# Autodesk Inventor assembly: 8_Omni-Directional_Wheel_217-2613
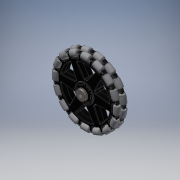
[picture p0: Inventor's stored thumbnail of the model, 180x180]
Saved by Autodesk Inventor 2018 (Build 220112000, 112)
## iProperties
Company: Microsoft
Created: 2012-12-03
Part Number: 8_Omni-Directional_Wheel_217-2613
Description: STEP AP203
Document SubType Name: Assembly
Designer: maste
Sending System: SolidWorks 2012
Preprocessor: SwSTEP 2.0
Title: 217-2613.20121203.STEP
Author: svradm
Revision Number: ANY
## Documents named in this file (12)
- C:\Users\maste\OneDrive\Documents\GitHub\2020CAD (offseason)\The Chad Kiwi\Part Files\8_Omni-Directional_Wheel_217-2613.iam
- C:\Users\maste\OneDrive\Documents\GitHub\2020CAD (offseason)\The Chad Kiwi\Part Files\217-2613-001 Rev1.ipt
- C:\Users\maste\OneDrive\Documents\GitHub\2020CAD (offseason)\The Chad Kiwi\Part Files\217-2613-003 Rev1.ipt
- C:\Users\maste\OneDrive\Documents\GitHub\2020CAD (offseason)\The Chad Kiwi\Part Files\217-2613-002 Rev1.ipt
- C:\Users\maste\OneDrive\Documents\GitHub\2020CAD (offseason)\The Chad Kiwi\Part Files\217-2613-004 Rev1.ipt
- C:\Users\maste\OneDrive\Documents\GitHub\2020CAD (offseason)\The Chad Kiwi\Part Files\BEAM-0750.ipt
- C:\Users\maste\OneDrive\Documents\GitHub\2020CAD (offseason)\The Chad Kiwi\Part Files\90116A020_90116A020.ipt
- C:\Users\maste\OneDrive\Documents\GitHub\2020CAD (offseason)\The Chad Kiwi\Part Files\217-2584-005 Rev1 A.ipt
- C:\Users\maste\OneDrive\Documents\GitHub\2020CAD (offseason)\The Chad Kiwi\Part Files\1_2_Hex_Bore_Aluminum_VersaHub_217-2592.ipt
- C:\Users\maste\OneDrive\Documents\GitHub\2020CAD (offseason)\The Chad Kiwi\Part Files\0.125 spacer.ipt
- C:\Users\maste\OneDrive\Documents\GitHub\2020CAD (offseason)\The Chad Kiwi\Part Files\0_500_Hex_ID_x_1_125_OD_x_0_313_WD_Flanged_Bearing_v2_217-3875.ipt
- C:\Users\maste\OneDrive\Documents\GitHub\2020CAD (offseason)\The Chad Kiwi\Part Files\am-1526 500Hex HD Collar Clamp (1).iam
## Components (114 placed, 113 different names)
1. 217-2613-001 Rev1_1
2. 217-2613-003 Rev1_2
3. 217-2613-002 Rev1_3 — Mate:4, Mate:5, Mate:6
4. 217-2613-001 Rev1_4
5. 217-2613-001 Rev1_5
6. 217-2613-001 Rev1_6
7. 217-2613-001 Rev1_7
8. 217-2613-001 Rev1_8
9. 217-2613-001 Rev1_9
10. 217-2613-001 Rev1_10
11. 217-2613-001 Rev1_11
12. 217-2613-001 Rev1_12
13. 217-2613-001 Rev1_13
14. 217-2613-001 Rev1_14
15. 217-2613-001 Rev1_15
16. 217-2613-001 Rev1_16
17. 217-2613-001 Rev1_17
18. 217-2613-001 Rev1_18
19. 217-2613-004 Rev1_19
20. 217-2613-004 Rev1_20
21. 217-2613-004 Rev1_21
22. 217-2613-004 Rev1_22
23. 217-2613-004 Rev1_23
24. 217-2613-004 Rev1_24
25. 217-2613-004 Rev1_25
26. 217-2613-004 Rev1_26
27. 217-2613-004 Rev1_27
28. 217-2613-004 Rev1_28
29. 217-2613-004 Rev1_29
30. 217-2613-004 Rev1_30
31. 217-2613-004 Rev1_31
32. 217-2613-004 Rev1_32
33. 217-2613-004 Rev1_33
34. 217-2613-004 Rev1_34
35. 217-2613-002 Rev1_35 — Mate:1, Mate:2, Mate:3
36. 217-2613-001 Rev1_36
37. 217-2613-004 Rev1_37
38. 217-2613-001 Rev1_38
39. 217-2613-001 Rev1_39
40. 217-2613-001 Rev1_40
41. 217-2613-001 Rev1_41
42. 217-2613-001 Rev1_42
43. 217-2613-001 Rev1_43
44. 217-2613-001 Rev1_44
45. 217-2613-001 Rev1_45
46. 217-2613-001 Rev1_46
47. 217-2613-001 Rev1_47
48. 217-2613-001 Rev1_48
49. 217-2613-001 Rev1_49
50. 217-2613-001 Rev1_50
51. 217-2613-001 Rev1_51
52. 217-2613-001 Rev1_52
53. 217-2613-004 Rev1_53
54. 217-2613-004 Rev1_54
55. 217-2613-004 Rev1_55
56. 217-2613-004 Rev1_56
57. 217-2613-004 Rev1_57
58. 217-2613-004 Rev1_58
59. 217-2613-004 Rev1_59
60. 217-2613-004 Rev1_60
61. 217-2613-004 Rev1_61
62. 217-2613-004 Rev1_62
63. 217-2613-004 Rev1_63
64. 217-2613-004 Rev1_64
65. 217-2613-004 Rev1_65
66. 217-2613-004 Rev1_66
67. 217-2613-004 Rev1_67
68. BEAM-0750_68
69. BEAM-0750_69
70. BEAM-0750_70
71. BEAM-0750_71
72. BEAM-0750_72
73. BEAM-0750_73
74. 90116A020_90116A020_74
75. 90116A020_90116A020_75
76. 90116A020_90116A020_76
77. 90116A020_90116A020_77
78. 90116A020_90116A020_78
79. 90116A020_90116A020_79
80. 90116A020_90116A020_80
81. 90116A020_90116A020_81
82. 90116A020_90116A020_82
83. 90116A020_90116A020_83
84. 90116A020_90116A020_84
85. 90116A020_90116A020_85
86. 90116A020_90116A020_86
87. 90116A020_90116A020_87
88. 90116A020_90116A020_88
89. 90116A020_90116A020_89
90. 90116A020_90116A020_90
91. 90116A020_90116A020_91
92. 90116A020_90116A020_92
93. 90116A020_90116A020_93
94. 90116A020_90116A020_94
95. 90116A020_90116A020_95
96. 90116A020_90116A020_96
97. 90116A020_90116A020_97
98. 90116A020_90116A020_98
99. 90116A020_90116A020_99
100. 90116A020_90116A020_100
101. 90116A020_90116A020_101
102. 90116A020_90116A020_102
103. 90116A020_90116A020_103
104. 90116A020_90116A020_104
105. 90116A020_90116A020_105
106. 217-2584-005 Rev1 A_106
107. 217-2584-005 Rev1 A_107
108. 217-2584-005 Rev1 A_108
109. 217-2584-005 Rev1 A_109
110. 1_2_Hex_Bore_Aluminum_VersaHub_217-2592:1 — Mate:1, Mate:2, Mate:3, Flush:1, Flush:2, Mate:7
111. 1_2_Hex_Bore_Aluminum_VersaHub_217-2592:2 — Mate:4, Mate:5, Mate:6, Flush:3, Flush:4, Mate:8
112. 0.125 spacer:1 — Flush:3, Flush:4, Mate:8, Flush:5, Flush:6, Mate:9
113. 0_500_Hex_ID_x_1_125_OD_x_0_313_WD_Flanged_Bearing_v2_217-3875:1 — Flush:5, Flush:6, Mate:9
114. am-1526 500Hex HD Collar Clamp (1):1 [sub-assembly] — Flush:1, Flush:2, Mate:7
## Relationships (15: Mate 9, Flush 6)
- Mate:1: 217-2613-002 Rev1_35 ↔ 1_2_Hex_Bore_Aluminum_VersaHub_217-2592:1
- Mate:2: 217-2613-002 Rev1_35 ↔ 1_2_Hex_Bore_Aluminum_VersaHub_217-2592:1
- Mate:3: 217-2613-002 Rev1_35 ↔ 1_2_Hex_Bore_Aluminum_VersaHub_217-2592:1
- Mate:4: 217-2613-002 Rev1_3 ↔ 1_2_Hex_Bore_Aluminum_VersaHub_217-2592:2
- Mate:5: 217-2613-002 Rev1_3 ↔ 1_2_Hex_Bore_Aluminum_VersaHub_217-2592:2
- Mate:6: 217-2613-002 Rev1_3 ↔ 1_2_Hex_Bore_Aluminum_VersaHub_217-2592:2
- Flush:1: 1_2_Hex_Bore_Aluminum_VersaHub_217-2592:1 ↔ am-1526 500Hex HD Collar Clamp (1):1
- Flush:2: 1_2_Hex_Bore_Aluminum_VersaHub_217-2592:1 ↔ am-1526 500Hex HD Collar Clamp (1):1
- Mate:7: 1_2_Hex_Bore_Aluminum_VersaHub_217-2592:1 ↔ am-1526 500Hex HD Collar Clamp (1):1
- Flush:3: 1_2_Hex_Bore_Aluminum_VersaHub_217-2592:2 ↔ 0.125 spacer:1
- Flush:4: 1_2_Hex_Bore_Aluminum_VersaHub_217-2592:2 ↔ 0.125 spacer:1
- Mate:8: 1_2_Hex_Bore_Aluminum_VersaHub_217-2592:2 ↔ 0.125 spacer:1
- Flush:5: 0.125 spacer:1 ↔ 0_500_Hex_ID_x_1_125_OD_x_0_313_WD_Flanged_Bearing_v2_217-3875:1
- Flush:6: 0.125 spacer:1 ↔ 0_500_Hex_ID_x_1_125_OD_x_0_313_WD_Flanged_Bearing_v2_217-3875:1
- Mate:9: 0.125 spacer:1 ↔ 0_500_Hex_ID_x_1_125_OD_x_0_313_WD_Flanged_Bearing_v2_217-3875:1
